# Autodesk Inventor assembly: 足ユニット
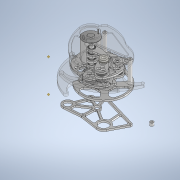
[picture p0: Inventor's stored thumbnail of the model, 180x180]
Saved by Autodesk Inventor 2022.2 (Build 262287010, 287A)
## iProperties
Created: 2022-01-10
Part Number: 足ユニット
Document SubType Name: Assembly
Designer: acps
Author: acps
## Documents named in this file (17)
- C:\Users\acps\Documents\srdc\srdc_ksh\脚\足ユニット.iam
- C:\Users\acps\Documents\srdc\srdc_ksh\脚\足(単独).iam
- C:\Users\acps\Documents\srdc\srdc_ksh\脚\足外フレーム.ipt
- C:\Users\acps\Documents\srdc\srdc_ksh\脚\足内フレーム.ipt
- C:\Users\acps\Documents\srdc\srdc_ksh\スペーサ\l40.ipt
- C:\Users\acps\Documents\srdc\srdc_ksh\カム\カム4.ipt
- C:\Users\acps\Documents\srdc\srdc_ksh\オイレス\w5f15-17n.ipt
- C:\Users\acps\Documents\srdc\srdc_ksh\モータ\M-RS-380.ipt
- C:\Users\acps\Documents\srdc\srdc_ksh\脚\ギア抑え.ipt
- C:\Users\acps\Documents\srdc\srdc_ksh\脚\モータマウント.ipt
- C:\Users\acps\Documents\srdc\srdc_ksh\ベアリング\Φ6-12a.ipt
- C:\Users\acps\Documents\srdc\srdc_ksh\スペーサ\l5.ipt
- C:\Users\acps\Documents\srdc\srdc_ksh\脚\ギア\初段_多段ギア.iam
- C:\Users\acps\Documents\srdc\srdc_ksh\脚\ギア\ぴにょん.ipt
- C:\Users\acps\Documents\srdc\srdc_ksh\ベアリング\M-φ4φ8a.ipt
- C:\Users\acps\Documents\srdc\srdc_ksh\ピン\φ4ピン　L20.ipt
- C:\Users\acps\Documents\srdc\srdc_ksh\ベアリング\φ4φ8ベアリングa.ipt
## Components (18 placed, 16 different names)
1. l40:1 — Insert:22
2. l40:2 — Insert:21, Insert:27
3. l40:3 — Mate:30, Insert:23, Mate:31
4. カム4:1 — Insert:9, Mate:33, Mate:34, Insert:24, Mate:37
5. w5f15-17n:1 — Insert:9, Mate:29
6. M-RS-380:1 — Mate:27, Insert:31, Mate:38, Insert:32
7. ギア抑え:1 — Mate:36, Mate:37
8. Φ6-12a:1 — Insert:28, Insert:29
9. l5:1
10. モータマウント:1 — Mate:35, Insert:30, Insert:31
11. 足内フレーム:1 — Mate:27, Mate:29, Insert:21, Insert:22, Mate:30, Insert:23, Mate:35, Insert:30, Mate:36, Mate:40, Insert:33, Insert:35
12. 足外フレーム:1 — Mate:32, Insert:27, Insert:28
13. 足(単独):1 [sub-assembly] — Mate:31, Mate:32, Mate:33, Mate:34, Insert:24, Insert:29
14. ぴにょん:1 — Mate:38, Insert:32
15. M-φ4φ8a:1 — Mate:40, Insert:33, Mate:41, Mate:42
16. 初段_多段ギア:1 [sub-assembly] — Mate:41
17. φ4ピン　L20:1 — Mate:42, Insert:35, Mate:43
18. φ4φ8ベアリングa:1 — Mate:43
## Relationships (28: Mate 15, Insert 13)
- Insert:9: カム4:1 ↔ w5f15-17n:1
- Mate:27: M-RS-380:1 ↔ 足内フレーム:1
- Mate:29: w5f15-17n:1 ↔ 足内フレーム:1
- Insert:21: l40:2 ↔ 足内フレーム:1
- Insert:22: l40:1 ↔ 足内フレーム:1
- Mate:30: l40:3 ↔ 足内フレーム:1
- Insert:23: l40:3 ↔ 足内フレーム:1
- Mate:31: l40:3 ↔ 足(単独):1
- Mate:32: 足外フレーム:1 ↔ 足(単独):1
- Mate:33: カム4:1 ↔ 足(単独):1
- Mate:34: カム4:1 ↔ 足(単独):1
- Insert:24: カム4:1 ↔ 足(単独):1
- Insert:27: l40:2 ↔ 足外フレーム:1
- Insert:28: Φ6-12a:1 ↔ 足外フレーム:1
- Insert:29: Φ6-12a:1 ↔ 足(単独):1
- Mate:35: モータマウント:1 ↔ 足内フレーム:1
- Insert:30: モータマウント:1 ↔ 足内フレーム:1
- Insert:31: M-RS-380:1 ↔ モータマウント:1
- Mate:36: ギア抑え:1 ↔ 足内フレーム:1
- Mate:37: カム4:1 ↔ ギア抑え:1
- Mate:38: M-RS-380:1 ↔ ぴにょん:1
- Insert:32: M-RS-380:1 ↔ ぴにょん:1
- Mate:40: 足内フレーム:1 ↔ M-φ4φ8a:1
- Insert:33: 足内フレーム:1 ↔ M-φ4φ8a:1
- Mate:41: M-φ4φ8a:1 ↔ 初段_多段ギア:1
- Mate:42: M-φ4φ8a:1 ↔ φ4ピン　L20:1
- Insert:35: 足内フレーム:1 ↔ φ4ピン　L20:1
- Mate:43: φ4ピン　L20:1 ↔ φ4φ8ベアリングa:1
